# Autodesk Inventor assembly: ENSAMBLE_CON_BRAZO
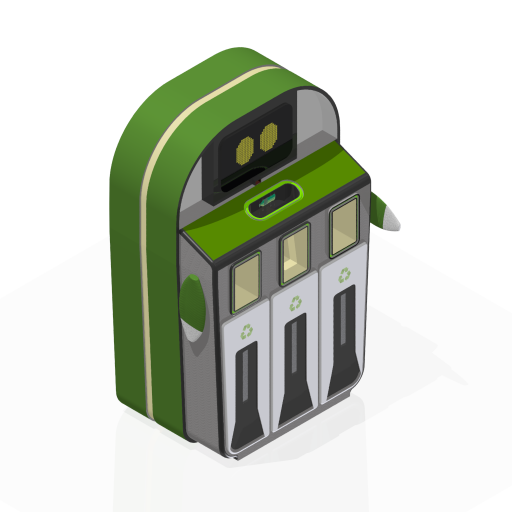
[picture p0: Inventor's stored thumbnail of the model, 512x512]
Saved by Autodesk Inventor 2024.3 (Build 283343000, 343)
## iProperties
Created: 2024-06-16
Part Number: ENSAMBLE_CON_BRAZO
Material: Generic
Document SubType Name: Assembly
Designer: Niler
Author: Niler
## Documents named in this file (3)
- C:\Users\Niler\OneDrive\Escritorio\RECICLADOR\RECICLADOR_MODELO_3D\VERSION_3\ENSAMBLE_CON_BRAZO.iam
- C:\Users\Niler\OneDrive\Escritorio\RECICLADOR\RECICLADOR_MODELO_3D\VERSION_3\CARCASA_V4 - Copy.ipt
- C:\Users\Niler\OneDrive\Escritorio\RECICLADOR\RECICLADOR_MODELO_3D\BRAZO.ipt
## Components (3 placed, 2 different names)
1. CARCASA_V4 - Copy:1 — Mate:1, Mate:2
2. BRAZO:1 — Mate:1
3. BRAZO:2 — Mate:2
## Relationships (2: Mate 2)
- Mate:1: CARCASA_V4 - Copy:1 ↔ BRAZO:1
- Mate:2: CARCASA_V4 - Copy:1 ↔ BRAZO:2
